# Autodesk Inventor assembly: Toughbox Mini Long Hex Output Shaft
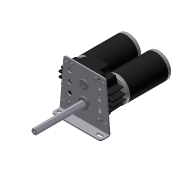
[picture p0: Inventor's stored thumbnail of the model, 180x180]
Saved by Autodesk Inventor 2011 (Build 150239000, 239)
## iProperties
Created: 2012-06-03
Part Number: Toughbox Mini Long Hex Output Shaft
Document SubType Name: Assembly
Designer: Nemo
Author: Nemo
## Documents named in this file (14)
- H:\Nemo\Documents\Robotics\COTS Parts\Gearboxes\Toughbox Mini Long Hex Output Shaft.iam
- H:\Nemo\Documents\Robotics\COTS Parts\Gearboxes\Housings\Toughbox Mini Housing.ipt
- H:\Nemo\Documents\Robotics\COTS Parts\Gearboxes\Bearings\Bearing R6zz.ipt
- H:\Nemo\Documents\Robotics\COTS Parts\Gearboxes\Shafts\Toughbox Long Hex Output Shaft.ipt
- H:\Nemo\Documents\Robotics\COTS Parts\Gearboxes\Shafts\Toughbox Small Hex Shaft.ipt
- H:\Nemo\Documents\Robotics\COTS Parts\Gearboxes\Gears\Gear 20dp 375hex 50T.ipt
- H:\Nemo\Documents\Robotics\COTS Parts\Gearboxes\Gears\Gear 20dp 375hex 14T.ipt
- H:\Nemo\Documents\Robotics\COTS Parts\Gearboxes\Housings\Toughbox Mini Plate.ipt
- H:\Nemo\Documents\Robotics\COTS Parts\Gearboxes\Bearings\Bearing FR8zz-hex.ipt
- H:\Nemo\Documents\Robotics\COTS Parts\Gearboxes\Bearings\Bearing FR6zz.ipt
- H:\Nemo\Documents\Robotics\COTS Parts\Gearboxes\Gears\Gear 20dp 500hex 50T.ipt
- H:\Nemo\Documents\Robotics\COTS Parts\Motors\CIM motor 12T.iam
- H:\Nemo\Documents\Robotics\COTS Parts\Fasteners\10-32 SHCS x625.ipt
- H:\Nemo\Documents\Robotics\COTS Parts\Fasteners\10-32 locknut.ipt
## Components (25 placed, 13 different names)
1. Toughbox Mini Housing:1 — Insert:1, Insert:2, Mate:5, Mate:6, Mate:7, Insert:7, Mate:8, Insert:8, Mate:9, Insert:10, Insert:12, Mate:10, Insert:13, Insert:14, Insert:19, Insert:20, Insert:21, Insert:22
2. Bearing R6zz:1 — Insert:2, Insert:4
3. Bearing R6zz:2 — Insert:1, Insert:3, Mate:2
4. Toughbox Long Hex Output Shaft:1 — Insert:4, Angle:3, Angle:4, Flush:1
5. Toughbox Cluster Shaft 375hex:1 — Insert:3, Mate:1, Angle:1, Mate:3, Angle:2
6. Gear 20dp 375hex 50T:1 — Mate:1, Angle:1, Mate:2, Mate:4
7. Gear 14T 20dp 375hex:1 — Mate:3, Angle:2, Mate:4
8. Toughbox Mini Plate:1 — Mate:5, Mate:6, Insert:5, Insert:6, Mate:10, Insert:15, Insert:16, Insert:17, Insert:18
9. Bearing FR8zz-hex:1 — Insert:5, Angle:3
10. Bearing FR6zz:1 — Insert:6
11. Gear 50T 20dp 500hex:1 — Mate:7, Angle:4, Flush:1
12. CIM motor 12T:1 [sub-assembly] — Insert:7, Mate:8
13. CIM motor 12T:2 [sub-assembly] — Insert:8, Mate:9
14. 10-32 SHCS x625:1 — Insert:13
15. 10-32 SHCS x625:2 — Insert:10
16. 10-32 SHCS x625:3 — Insert:14
17. 10-32 SHCS x625:4 — Insert:12
18. 10-32 SHCS x625:5 — Insert:15
19. 10-32 SHCS x625:6 — Insert:16
20. 10-32 SHCS x625:7 — Insert:17
21. 10-32 SHCS x625:8 — Insert:18
22. 10-32 locknut:1 — Insert:19
23. 10-32 locknut:2 — Insert:20
24. 10-32 locknut:3 — Insert:21
25. 10-32 locknut:4 — Insert:22
## Relationships (35: Insert 20, Mate 10, Angle 4, Flush 1)
- Insert:1: Toughbox Mini Housing:1 ↔ Bearing R6zz:2
- Insert:2: Toughbox Mini Housing:1 ↔ Bearing R6zz:1
- Insert:3: Bearing R6zz:2 ↔ Toughbox Cluster Shaft 375hex:1
- Mate:1: Toughbox Cluster Shaft 375hex:1 ↔ Gear 20dp 375hex 50T:1
- Angle:1 (0 deg): Toughbox Cluster Shaft 375hex:1 ↔ Gear 20dp 375hex 50T:1
- Mate:2: Bearing R6zz:2 ↔ Gear 20dp 375hex 50T:1
- Mate:3: Toughbox Cluster Shaft 375hex:1 ↔ Gear 14T 20dp 375hex:1
- Angle:2 (0 deg): Toughbox Cluster Shaft 375hex:1 ↔ Gear 14T 20dp 375hex:1
- Mate:4: Gear 20dp 375hex 50T:1 ↔ Gear 14T 20dp 375hex:1
- Insert:4: Bearing R6zz:1 ↔ Toughbox Long Hex Output Shaft:1
- Mate:5: Toughbox Mini Housing:1 ↔ Toughbox Mini Plate:1
- Mate:6: Toughbox Mini Housing:1 ↔ Toughbox Mini Plate:1
- Insert:5: Toughbox Mini Plate:1 ↔ Bearing FR8zz-hex:1
- Angle:3 (0 deg): Toughbox Long Hex Output Shaft:1 ↔ Bearing FR8zz-hex:1
- Insert:6: Toughbox Mini Plate:1 ↔ Bearing FR6zz:1
- Mate:7: Toughbox Mini Housing:1 ↔ Gear 50T 20dp 500hex:1
- Angle:4 (0 deg): Toughbox Long Hex Output Shaft:1 ↔ Gear 50T 20dp 500hex:1
- Flush:1: Toughbox Long Hex Output Shaft:1 ↔ Gear 50T 20dp 500hex:1
- Insert:7: Toughbox Mini Housing:1 ↔ CIM motor 12T:1
- Mate:8: Toughbox Mini Housing:1 ↔ CIM motor 12T:1
- Insert:8: Toughbox Mini Housing:1 ↔ CIM motor 12T:2
- Mate:9: Toughbox Mini Housing:1 ↔ CIM motor 12T:2
- Insert:10: Toughbox Mini Housing:1 ↔ 10-32 SHCS x625:2
- Insert:12: Toughbox Mini Housing:1 ↔ 10-32 SHCS x625:4
- Mate:10: Toughbox Mini Housing:1 ↔ Toughbox Mini Plate:1
- Insert:13: Toughbox Mini Housing:1 ↔ 10-32 SHCS x625:1
- Insert:14: Toughbox Mini Housing:1 ↔ 10-32 SHCS x625:3
- Insert:15: Toughbox Mini Plate:1 ↔ 10-32 SHCS x625:5
- Insert:16: Toughbox Mini Plate:1 ↔ 10-32 SHCS x625:6
- Insert:17: Toughbox Mini Plate:1 ↔ 10-32 SHCS x625:7
- Insert:18: Toughbox Mini Plate:1 ↔ 10-32 SHCS x625:8
- Insert:19: Toughbox Mini Housing:1 ↔ 10-32 locknut:1
- Insert:20: Toughbox Mini Housing:1 ↔ 10-32 locknut:2
- Insert:21: Toughbox Mini Housing:1 ↔ 10-32 locknut:3
- Insert:22: Toughbox Mini Housing:1 ↔ 10-32 locknut:4
